# Autodesk Inventor assembly: antenna_assemb
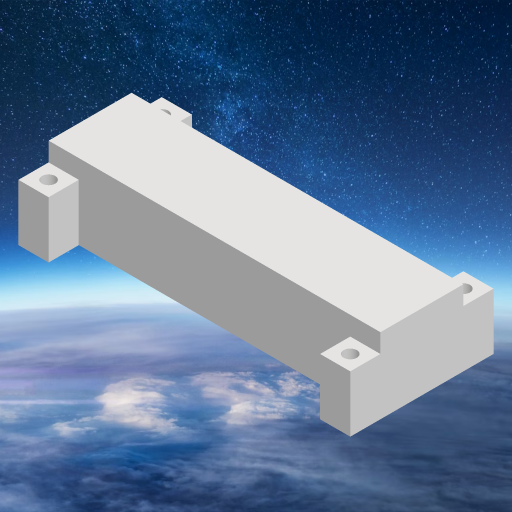
[picture p0: Inventor's stored thumbnail of the model, 512x512]
Saved by Autodesk Inventor 2023 (Build 270158000, 158)
## iProperties
Created: 2023-10-30
Part Number: antenna_assemb
Document SubType Name: Assembly
Designer: 310611102
Author: 310611102
## Documents named in this file (4)
- C:\Users\310611102\Documents\Inventor\SSR\avionics_2023ver\assembly\antenna_assemb.iam
- C:\Users\310611102\Documents\Inventor\SSR\avionics_2023ver\electronics\stick_antenna_case.ipt
- C:\Users\310611102\Documents\Inventor\SSR\avionics_2023ver\electronics\stick_antenna_434MHz.ipt
- C:\Users\310611102\Documents\Inventor\SSR\avionics_2023ver\electronics\stick_antenna__case_cap.ipt
## Components (3 placed, 3 different names)
1. stick_antenna_case:1 — Insert:1, Insert:2, Insert:3
2. stick_antenna_434MHz:1 — Insert:1
3. stick_antenna__case_cap:1 — Insert:2, Insert:3
## Relationships (3: Insert 3)
- Insert:1: stick_antenna_case:1 ↔ stick_antenna_434MHz:1
- Insert:2: stick_antenna_case:1 ↔ stick_antenna__case_cap:1
- Insert:3: stick_antenna_case:1 ↔ stick_antenna__case_cap:1
